# Autodesk Inventor assembly: ENSAMBLE_NUEVA_CREMALLERA
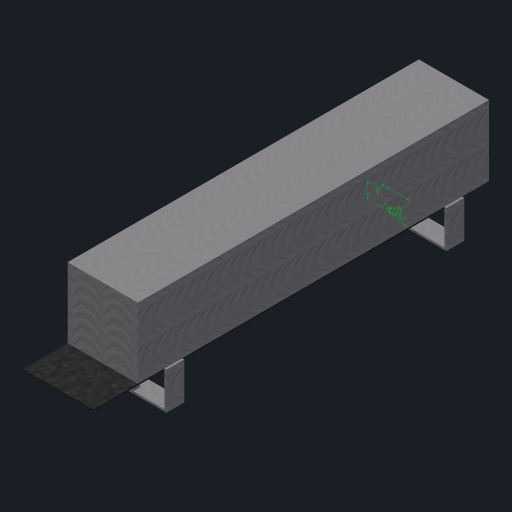
[picture p0: Inventor's stored thumbnail of the model, 512x512]
Saved by Autodesk Inventor 2024.3 (Build 283343000, 343)
## iProperties
Created: 2024-08-24
Part Number: ENSAMBLE_NUEVA_CREMALLERA
Material: Generic
Document SubType Name: Assembly
Designer: Niler
Author: Niler
## Documents named in this file (6)
- C:\Users\Niler\OneDrive\Escritorio\RECICLADOR\RECICLADOR_MODELO_3D\NUEVA CREMALLERA\ENSAMBLE_NUEVA_CREMALLERA.iam
- C:\Users\Niler\OneDrive\Escritorio\RECICLADOR\RECICLADOR_MODELO_3D\NUEVA CREMALLERA\TUBO.ipt
- C:\Users\Niler\OneDrive\Escritorio\RECICLADOR\RECICLADOR_MODELO_3D\NUEVA CREMALLERA\DESLIZANTE.ipt
- C:\Users\Niler\OneDrive\Escritorio\RECICLADOR\RECICLADOR_MODELO_3D\NUEVA CREMALLERA\APOYO_PLETINA.ipt
- C:\Users\Niler\OneDrive\Escritorio\RECICLADOR\RECICLADOR_MODELO_3D\NUEVA CREMALLERA\PARA_TUERCA.ipt
- C:\Users\Niler\OneDrive\Escritorio\RECICLADOR\RECICLADOR_MODELO_3D\NUEVA CREMALLERA\OTRO_EXTREMO.ipt
## Components (6 placed, 5 different names)
1. TUBO:1 — Flush:1, Mate:1, Mate:2, Mate:3, Mate:4, Mate:5
2. DESLIZANTE:1 — Flush:1, Mate:1, Flush:2, Mate:6, Flush:3
3. APOYO_PLETINA:1 — Mate:2, Mate:3, Mate:7, Flush:4
4. APOYO_PLETINA:2 — Mate:4, Mate:5
5. PARA_TUERCA:1 — Flush:2, Mate:6, Flush:3
6. OTRO_EXTREMO:1 — Mate:7, Flush:4
## Relationships (11: Mate 7, Flush 4)
- Flush:1: TUBO:1 ↔ DESLIZANTE:1
- Mate:1: TUBO:1 ↔ DESLIZANTE:1
- Mate:2: TUBO:1 ↔ APOYO_PLETINA:1
- Mate:3: TUBO:1 ↔ APOYO_PLETINA:1
- Mate:4: TUBO:1 ↔ APOYO_PLETINA:2
- Mate:5: TUBO:1 ↔ APOYO_PLETINA:2
- Flush:2 (20 mm): DESLIZANTE:1 ↔ PARA_TUERCA:1
- Mate:6: DESLIZANTE:1 ↔ PARA_TUERCA:1
- Flush:3: DESLIZANTE:1 ↔ PARA_TUERCA:1
- Mate:7: APOYO_PLETINA:1 ↔ OTRO_EXTREMO:1
- Flush:4: APOYO_PLETINA:1 ↔ OTRO_EXTREMO:1
